# Autodesk Inventor assembly: Полый вал
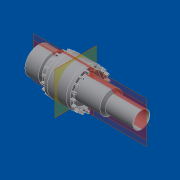
[picture p0: Inventor's stored thumbnail of the model, 180x180]
Saved by Autodesk Inventor 2016 SP1 (Build 200210100, 210)
## iProperties
Created: 2016-05-15
Part Number: Полый вал
Material: Типовые
Document SubType Name: Assembly
Designer: AS
Author: AS
## Documents named in this file (3)
- D:\Дела Алексея\Мехатронный узел - модель R2\Полый вал.iam
- D:\Дела Алексея\Мехатронный узел - модель R2\Полый вал.ipt
- D:\Дела Алексея\Мехатронный узел - модель R2\Сердечник ротора.ipt
## Components (2 placed, 2 different names)
1. Полый вал:1 — Совмещение:1, Совмещение:3, Заподлицо:1, Совмещение:4, Заподлицо:3
2. Сердечник ротора:1 — Совмещение:3, Заподлицо:1, Совмещение:4, Заподлицо:2
## Relationships (6: Mate 3, Flush 3)
- Совмещение:1 [Mate]: Полый вал:1
- Совмещение:3 [Mate]: Полый вал:1 ↔ Сердечник ротора:1
- Заподлицо:1 [Flush]: Полый вал:1 ↔ Сердечник ротора:1
- Совмещение:4 [Mate]: Полый вал:1 ↔ Сердечник ротора:1
- Заподлицо:2 [Flush]: Сердечник ротора:1
- Заподлицо:3 [Flush]: Полый вал:1
